# Autodesk Inventor assembly: Arms-with-motor
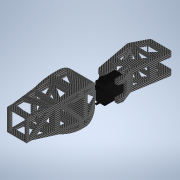
[picture p0: Inventor's stored thumbnail of the model, 180x180]
Saved by Autodesk Inventor 2022 (Build 260153000, 153)
## iProperties
Created: 2022-04-26
Part Number: Arms-with-motor
Document SubType Name: Assembly
Designer: dirks
Author: dirks
## Documents named in this file (4)
- C:\Users\dirks\Arny-de-humanoid-robot\Parts\Tests\Arms-with-motor.iam
- C:\Users\dirks\Arny-de-humanoid-robot\Parts\Onderarm(en).ipt
- C:\Users\dirks\Arny-de-humanoid-robot\Parts\Upper-Arm.ipt
- C:\Users\dirks\Arny-de-humanoid-robot\Parts\Imported Components\SERVO motor\Servo MOtor.ipt
## Components (3 placed, 3 different names)
1. Onderarm(en):1
2. Upper-Arm:1 — Mate:1, Mate:2, Mate:3
3. Servo MOtor:1 — Mate:1, Mate:2, Mate:3
## Relationships (3: Mate 3)
- Mate:1: Upper-Arm:1 ↔ Servo MOtor:1
- Mate:2: Upper-Arm:1 ↔ Servo MOtor:1
- Mate:3 (0.2 mm): Upper-Arm:1 ↔ Servo MOtor:1
